# Autodesk Inventor assembly: bearing_abec7
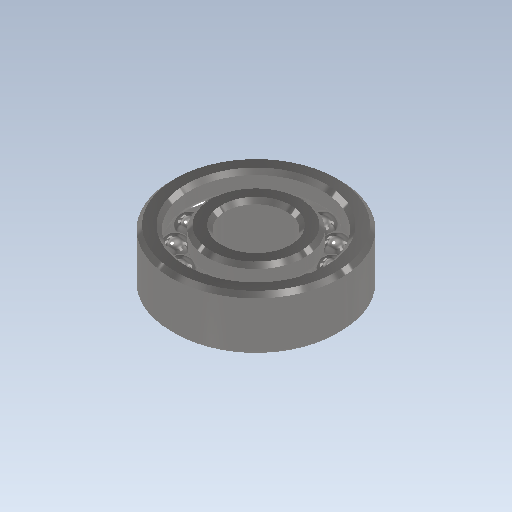
[picture p0: Inventor's stored thumbnail of the model, 512x512]
Saved by Autodesk Inventor 2020.1 (Build 241239000, 239)
## iProperties
Created: 2018-11-23
Part Number: bearing_abec7
Document SubType Name: Assembly
Designer: Petar
Mass: 13.4781 g
Surface Area: 21.8074 cm^2
Volume: 1.68476 cm^3
Density: 8 g/cm^3
Author: Petar
## Documents named in this file (3)
- D:\OMG\E-Board\CAD\Inventor\Trucks\Bearings\bearing_abec7.iam
- D:\OMG\E-Board\CAD\Inventor\Trucks\Bearings\bearing_in.ipt
- D:\OMG\E-Board\CAD\Inventor\Trucks\Bearings\bearing_out.ipt
## Components (2 placed, 2 different names)
1. bearing_in:1 — Insert:1
2. bearing_out:1 — Insert:1
## Relationships (1: Insert 1)
- Insert:1: bearing_in:1 ↔ bearing_out:1
